# Autodesk Inventor assembly: ASY MSC 200 BACK
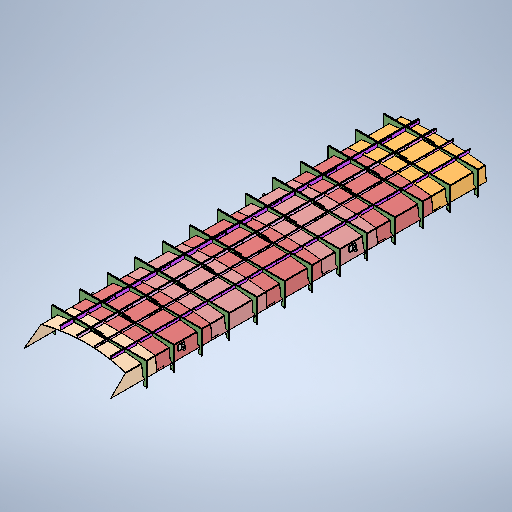
[picture p0: Inventor's stored thumbnail of the model, 512x512]
Saved by Autodesk Inventor 2025.1 (Build 291241020, 241B)
## iProperties
Created: 2024-07-19
Part Number: ASY MSC 200 BACK
Document SubType Name: Assembly
Designer: pokla
Stock Number: ASY МОО 200 спина
Mass: 379257 g
Surface Area: 351509 cm^2
Volume: 47407.1 cm^3
Density: 8 g/cm^3
Author: pokla
## Documents named in this file (11)
- C:\Users\user\YandexDisk-badmisterfox\домашниий пк\Inventor\Manturovo\Manturovo_Se-clar\ASY MSC 200 BACK.iam
- C:\Users\user\YandexDisk-badmisterfox\домашниий пк\Inventor\Manturovo\Manturovo_Se-clar\MSC 201 sheet back basic.ipt
- C:\Users\user\YandexDisk-badmisterfox\домашниий пк\Inventor\Manturovo\Manturovo_Se-clar\MSC 203 rib back.ipt
- C:\Users\user\YandexDisk-badmisterfox\домашниий пк\Inventor\Manturovo\Manturovo_Se-clar\MSC 202 BACK-neck.ipt
- C:\Users\user\YandexDisk-badmisterfox\домашниий пк\Inventor\Manturovo\Manturovo_Se-clar\MSC 205 stringer back ^.ipt
- C:\Users\user\YandexDisk-badmisterfox\домашниий пк\Inventor\Manturovo\Manturovo_Se-clar\MSC 206 stringer back ^^.ipt
- C:\Users\user\YandexDisk-badmisterfox\домашниий пк\Inventor\Manturovo\Manturovo_Se-clar\MSC 208 sheet back mould.ipt
- C:\Users\user\YandexDisk-badmisterfox\домашниий пк\Inventor\Manturovo\Manturovo_Se-clar\MSC 204 stringer back ^.ipt
- C:\Users\user\YandexDisk-badmisterfox\домашниий пк\Inventor\Manturovo\Manturovo_Se-clar\MSC 207 stringer back ^^.ipt
- C:\Users\user\YandexDisk-badmisterfox\домашниий пк\Inventor\Manturovo\Manturovo_Se-clar\MSC 208 sheet back START.ipt
- C:\Users\user\YandexDisk-badmisterfox\домашниий пк\Inventor\Manturovo\Manturovo_Se-clar\ASY MSC D-ring.iam
## Components (78 placed, 10 different names)
1. MSC 201 sheet back basic.ipt:1 — Mate:1, Flush:2, Tangent:2, Rigid:65, Rigid:84, Mate:2, Mate:3, Flush:3
2. MSC 201 sheet back basic.ipt:2 — Rigid:65, Rigid:66, Flush:5, Flush:7
3. MSC 201 sheet back basic.ipt:3 — Rigid:66, Rigid:67
4. MSC 202 BACK-neck.ipt:1 — Rigid:69
5. MSC 201 sheet back basic.ipt:4 — Rigid:68, Rigid:69, Flush:4, Flush:8
6. MSC 201 sheet back basic.ipt:5 — Rigid:67, Rigid:68
7. MSC 208 sheet back START:1 — Rigid:84
8. MSC 205 stringer back ^.ipt:1 — Rigid:75, Rigid:76, Rigid:80
9. MSC 205 stringer back ^.ipt:2 — Rigid:77, Rigid:81
10. MSC 206 stringer back ^^.ipt:1 — Rigid:78, Rigid:82
11. MSC 206 stringer back ^^.ipt:2 — Rigid:79, Rigid:83
12. MSC 203 rib back.ipt:1 — Rigid:70, Rigid:73, Mate:3
13. MSC 203 rib back.ipt:2 — Rigid:70, Mate:2
14. ASY MSC D-ring:4 [sub-assembly] — Flush:4, Mate:8, Flush:9
15. ASY MSC D-ring:3 [sub-assembly] — Flush:5, Mate:9, Flush:6
16. ASY MSC D-ring:2 [sub-assembly] — Flush:6, Flush:7
17. ASY MSC D-ring:1 [sub-assembly] — Flush:8, Flush:9
18. MSC 204 stringer back ^.ipt:1 — Rigid:80
19. MSC 204 stringer back ^.ipt:2 — Rigid:81
20. MSC 207 stringer back ^^.ipt:1 — Rigid:82
21. MSC 207 stringer back ^^.ipt:2 — Rigid:83
22. MSC 208 sheet back mould.ipt:1 — Mate:1, Flush:2, Tangent:2, Rigid:22, Rigid:23
23. MSC 208 sheet back mould.ipt:2 — Rigid:22, Rigid:25
24. MSC 208 sheet back mould.ipt:3 — Rigid:23, Rigid:24
25. MSC 208 sheet back mould.ipt:4 — Rigid:24
26. MSC 208 sheet back mould.ipt:5 — Rigid:25, Rigid:27
27. MSC 208 sheet back mould.ipt:6 — Rigid:27
28. MSC 208 sheet back mould.ipt:7 — Rigid:31
29. MSC 208 sheet back mould.ipt:8 — Rigid:31
30. MSC 208 sheet back mould.ipt:9
31. MSC 208 sheet back mould.ipt:10
32. MSC 208 sheet back mould.ipt:11 — Rigid:33
33. MSC 208 sheet back mould.ipt:12 — Rigid:33
34. MSC 208 sheet back mould.ipt:13
35. MSC 203 rib back.ipt:3 — Rigid:73, Rigid:74, Rigid:78
36. MSC 203 rib back.ipt:4 — Rigid:74, Rigid:77, Rigid:79
37. MSC 203 rib back.ipt:5 — Rigid:75
38. MSC 203 rib back.ipt:6
39. MSC 203 rib back.ipt:7
40. MSC 203 rib back.ipt:8
41. MSC 203 rib back.ipt:9
42. MSC 203 rib back.ipt:10 — Mate:9
43. MSC 203 rib back.ipt:11
44. MSC 203 rib back.ipt:12
45. MSC 203 rib back.ipt:13
46. MSC 203 rib back.ipt:14
47. MSC 203 rib back.ipt:15
48. MSC 203 rib back.ipt:16
49. MSC 203 rib back.ipt:17
50. MSC 203 rib back.ipt:18
51. MSC 203 rib back.ipt:19
52. MSC 203 rib back.ipt:20
53. MSC 203 rib back.ipt:21
54. MSC 203 rib back.ipt:22
55. MSC 203 rib back.ipt:23
56. MSC 203 rib back.ipt:24 — Mate:8
57. MSC 203 rib back.ipt:25
58. MSC 203 rib back.ipt:26
59. MSC 206 stringer back ^^.ipt:3
60. MSC 205 stringer back ^.ipt:3 — Rigid:76
61. MSC 205 stringer back ^.ipt:4
62. MSC 206 stringer back ^^.ipt:4 — Flush:3
63. MSC 206 stringer back ^^.ipt:5
64. MSC 205 stringer back ^.ipt:5
65. MSC 205 stringer back ^.ipt:6
66. MSC 206 stringer back ^^.ipt:6
67. MSC 206 stringer back ^^.ipt:7
68. MSC 205 stringer back ^.ipt:7
69. MSC 205 stringer back ^.ipt:8
70. MSC 206 stringer back ^^.ipt:8
71. MSC 206 stringer back ^^.ipt:9
72. MSC 205 stringer back ^.ipt:9
73. MSC 205 stringer back ^.ipt:10
74. MSC 206 stringer back ^^.ipt:10
75. MSC 206 stringer back ^^.ipt:11
76. MSC 205 stringer back ^.ipt:11
77. MSC 205 stringer back ^.ipt:12
78. MSC 206 stringer back ^^.ipt:12
## Component patterns: (12 elements, first: MSC 203 rib back.ipt:3 + MSC 203 rib back.ipt:4), (5 elements, first: MSC 206 stringer back ^^.ipt:3 + MSC 205 stringer back ^.ipt:3 + MSC 205 stringer back ^.ipt:4 + MSC 206 stringer back ^^.ipt:4)
## Relationships (51: WeldJoint 33, Mate 9, Flush 8, Tangent 1)
- [WeldJoint]: MSC 205 stringer back ^.ipt:2 ↔ MSC 205 stringer back ^.ipt:4
- [WeldJoint]: MSC 206 stringer back ^^.ipt:1 ↔ MSC 206 stringer back ^^.ipt:3
- [WeldJoint]: MSC 206 stringer back ^^.ipt:2 ↔ MSC 206 stringer back ^^.ipt:4
- Mate:1: MSC 201 sheet back basic.ipt:1 ↔ MSC 208 sheet back mould.ipt:1
- Flush:2 (248.5 mm): MSC 201 sheet back basic.ipt:1 ↔ MSC 208 sheet back mould.ipt:1
- Tangent:2: MSC 201 sheet back basic.ipt:1 ↔ MSC 208 sheet back mould.ipt:1
- Rigid:22 [WeldJoint] (497 mm): MSC 208 sheet back mould.ipt:1 ↔ MSC 208 sheet back mould.ipt:2
- Rigid:23 [WeldJoint] (497 mm): MSC 208 sheet back mould.ipt:1 ↔ MSC 208 sheet back mould.ipt:3
- Rigid:24 [WeldJoint] (497 mm): MSC 208 sheet back mould.ipt:3 ↔ MSC 208 sheet back mould.ipt:4
- Rigid:25 [WeldJoint] (497 mm): MSC 208 sheet back mould.ipt:2 ↔ MSC 208 sheet back mould.ipt:5
- [WeldJoint] (497 mm): MSC 208 sheet back mould.ipt:6 ↔ MSC 208 sheet back mould.ipt:7
- Rigid:27 [WeldJoint] (497 mm): MSC 208 sheet back mould.ipt:5 ↔ MSC 208 sheet back mould.ipt:6
- [WeldJoint] (497 mm): MSC 208 sheet back mould.ipt:8 ↔ MSC 208 sheet back mould.ipt:9
- [WeldJoint] (497 mm): MSC 208 sheet back mould.ipt:10 ↔ MSC 208 sheet back mould.ipt:11
- [WeldJoint] (497 mm): MSC 208 sheet back mould.ipt:9 ↔ MSC 208 sheet back mould.ipt:10
- Rigid:31 [WeldJoint] (497 mm): MSC 208 sheet back mould.ipt:7 ↔ MSC 208 sheet back mould.ipt:8
- [WeldJoint] (497 mm): MSC 208 sheet back mould.ipt:12 ↔ MSC 208 sheet back mould.ipt:13
- Rigid:33 [WeldJoint] (497 mm): MSC 208 sheet back mould.ipt:11 ↔ MSC 208 sheet back mould.ipt:12
- Rigid:65 [WeldJoint]: MSC 201 sheet back basic.ipt:1 ↔ MSC 201 sheet back basic.ipt:2
- Rigid:66 [WeldJoint]: MSC 201 sheet back basic.ipt:2 ↔ MSC 201 sheet back basic.ipt:3
- Rigid:67 [WeldJoint]: MSC 201 sheet back basic.ipt:3 ↔ MSC 201 sheet back basic.ipt:5
- Rigid:68 [WeldJoint]: MSC 201 sheet back basic.ipt:4 ↔ MSC 201 sheet back basic.ipt:5
- Rigid:69 [WeldJoint]: MSC 202 BACK-neck.ipt:1 ↔ MSC 201 sheet back basic.ipt:4
- Rigid:70 [WeldJoint] (-100 mm): MSC 203 rib back.ipt:1 ↔ MSC 203 rib back.ipt:2
- Rigid:73 [WeldJoint] (-490 mm): MSC 203 rib back.ipt:1 ↔ MSC 203 rib back.ipt:3
- Rigid:74 [WeldJoint] (-100 mm): MSC 203 rib back.ipt:3 ↔ MSC 203 rib back.ipt:4
- Rigid:75 [WeldJoint] (2 mm): MSC 205 stringer back ^.ipt:1 ↔ MSC 203 rib back.ipt:5
- Rigid:76 [WeldJoint]: MSC 205 stringer back ^.ipt:1 ↔ MSC 205 stringer back ^.ipt:3
- Rigid:77 [WeldJoint] (2 mm): MSC 205 stringer back ^.ipt:2 ↔ MSC 203 rib back.ipt:4
- Rigid:78 [WeldJoint] (2 mm): MSC 206 stringer back ^^.ipt:1 ↔ MSC 203 rib back.ipt:3
- Rigid:79 [WeldJoint]: MSC 206 stringer back ^^.ipt:2 ↔ MSC 203 rib back.ipt:4
- Rigid:80 [WeldJoint]: MSC 205 stringer back ^.ipt:1 ↔ MSC 204 stringer back ^.ipt:1
- Rigid:81 [WeldJoint]: MSC 205 stringer back ^.ipt:2 ↔ MSC 204 stringer back ^.ipt:2
- Rigid:82 [WeldJoint]: MSC 206 stringer back ^^.ipt:1 ↔ MSC 207 stringer back ^^.ipt:1
- Rigid:83 [WeldJoint]: MSC 206 stringer back ^^.ipt:2 ↔ MSC 207 stringer back ^^.ipt:2
- Rigid:84 [WeldJoint]: MSC 201 sheet back basic.ipt:1 ↔ MSC 208 sheet back START:1
- Mate:2: MSC 201 sheet back basic.ipt:1 ↔ MSC 203 rib back.ipt:2
- Mate:3: MSC 201 sheet back basic.ipt:1 ↔ MSC 203 rib back.ipt:1
- Flush:3 (490 mm): MSC 201 sheet back basic.ipt:1 ↔ MSC 206 stringer back ^^.ipt:4
- [Mate]: MSC 201 sheet back basic.ipt:4 ↔ ASY MSC D-ring:1
- [Mate]: MSC 201 sheet back basic.ipt:2 ↔ ASY MSC D-ring:2
- [Mate]: MSC 201 sheet back basic.ipt:5 ↔ ASY MSC D-ring:4
- [Mate]: MSC 201 sheet back basic.ipt:2 ↔ ASY MSC D-ring:3
- Flush:4 (-115 mm): MSC 201 sheet back basic.ipt:4 ↔ ASY MSC D-ring:4
- Mate:8 (140 mm): ASY MSC D-ring:4 ↔ MSC 203 rib back.ipt:24
- Flush:5 (-115 mm): MSC 201 sheet back basic.ipt:2 ↔ ASY MSC D-ring:3
- Mate:9 (125 mm): ASY MSC D-ring:3 ↔ MSC 203 rib back.ipt:10
- Flush:6: ASY MSC D-ring:3 ↔ ASY MSC D-ring:2
- Flush:7 (-115 mm): MSC 201 sheet back basic.ipt:2 ↔ ASY MSC D-ring:2
- Flush:8 (-115 mm): MSC 201 sheet back basic.ipt:4 ↔ ASY MSC D-ring:1
- Flush:9: ASY MSC D-ring:4 ↔ ASY MSC D-ring:1
## Named parameters: d42_d41 = 497 mm, d44_d41 = 497 mm, d45_d42_d41 = 497 mm, d46_d43 = 497 mm, d48_d45_d42_d41 = 497 mm
